# Autodesk Inventor assembly: X Axis
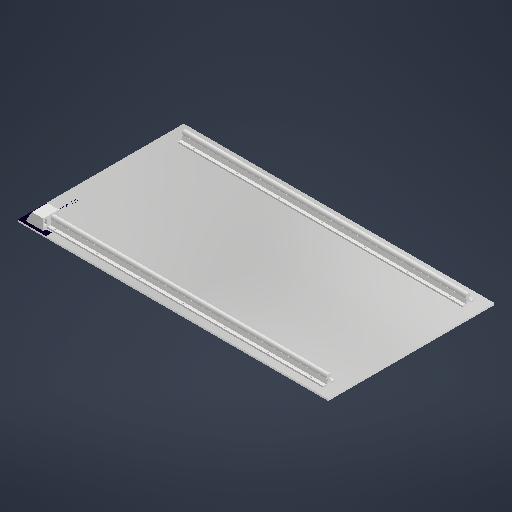
[picture p0: Inventor's stored thumbnail of the model, 512x512]
Saved by Autodesk Inventor 2025.1 (Build 291241000, 241)
## iProperties
Created: 2024-11-25
Part Number: X Axis
Document SubType Name: Assembly
Designer: jerem
Author: jerem
## Documents named in this file (5)
- C:\Users\jerem\Documents\GitHub\Perovskite-Automated-Synthesis-System\CAD\Gantry\X Axis.iam
- C:\Users\jerem\Documents\GitHub\Perovskite-Automated-Synthesis-System\CAD\Non 3D Printed Parts\Base Plate.ipt
- C:\Users\jerem\Documents\GitHub\Perovskite-Automated-Synthesis-System\CAD\Non 3D Printed Parts\Linear Rails\Linear Rail.ipt
- C:\Users\jerem\Documents\GitHub\Perovskite-Automated-Synthesis-System\CAD\Gantry\X Axis End.ipt
- C:\Users\jerem\Documents\GitHub\Perovskite-Automated-Synthesis-System\CAD\Non 3D Printed Parts\Bearings\13mmOD Belt Bearing Half.ipt
## Components (6 placed, 4 different names)
1. Base Plate:1
2. Linear Rail:1 — Mate:4, Mate:5, Mate:6
3. Linear Rail:2
4. X Axis End:1 — Mate:4, Mate:5, Mate:6, Mate:9
5. 13mmOD Belt Bearing Half:1 — Mate:7, Mate:8
6. 13mmOD Belt Bearing Half:2 — Mate:7, Mate:8, Mate:9
## Relationships (12: Mate 9, Flush 3)
- [Flush] (50 mm): Base Plate:1 ↔ Linear Rail:1
- [Flush] (25 mm): Base Plate:1 ↔ Linear Rail:1
- [Mate]: Base Plate:1 ↔ Linear Rail:1
- [Mate]: Base Plate:1 ↔ Linear Rail:2
- [Flush]: Linear Rail:1 ↔ Linear Rail:2
- [Mate] (450 mm): Linear Rail:1 ↔ Linear Rail:2
- Mate:4: Linear Rail:1 ↔ X Axis End:1
- Mate:5: Linear Rail:1 ↔ X Axis End:1
- Mate:6: Linear Rail:1 ↔ X Axis End:1
- Mate:7: 13mmOD Belt Bearing Half:1 ↔ 13mmOD Belt Bearing Half:2
- Mate:8: 13mmOD Belt Bearing Half:1 ↔ 13mmOD Belt Bearing Half:2
- Mate:9: X Axis End:1 ↔ 13mmOD Belt Bearing Half:2
